# Autodesk Inventor assembly: RightMecanum-SubAssem01_MIR1
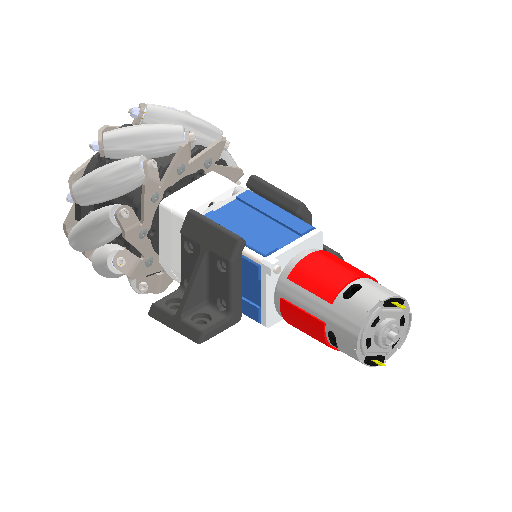
[picture p0: Inventor's stored thumbnail of the model, 512x512]
Saved by Autodesk Inventor 2024.1 (Build 281209000, 209)
## iProperties
Created: 2022-07-11
Part Number: RightMecanum-SubAssem01_MIR1
Document SubType Name: Assembly
Designer: dbt5238
Author: Dave
## Documents named in this file (9)
- E:\ChalkbotMechanical\Chalkbot1.0\Chassis\V1\RightMecanum-SubAssem01_MIR1.iam
- E:\ChalkbotMechanical\Chalkbot1.0\Chassis\V1\Motor and Gearbox STEP files\2 Stage HD - 57 Sport_MIR1.ipt
- E:\ChalkbotMechanical\Chalkbot1.0\Chassis\V1\Mechanum STEP files\am-3775a AndyMark RedLine Motor (1)_MIR1.ipt
- E:\ChalkbotMechanical\Chalkbot1.0\Chassis\V1\Motor and Gearbox STEP files\Hex Bore Mag Encoder Housing (217-6785)_MIR1.iam
- E:\ChalkbotMechanical\Chalkbot1.0\Chassis\V1\Motor and Gearbox STEP files\am-3791 - 3000 x 500 Hex Shaft_MIR1.ipt
- E:\ChalkbotMechanical\Chalkbot1.0\Chassis\V1\Motor Mounts_MIR1.ipt
- E:\ChalkbotMechanical\Chalkbot1.0\Chassis\V1\Shaft Spacers V2_MIR1.ipt
- E:\ChalkbotMechanical\Chalkbot1.0\Chassis\V1\Mechanum STEP files\am-3918L 4HD 500H Mecanum Right_MIR1.iam
- E:\ChalkbotMechanical\Chalkbot1.0\Chassis\V1\Motor and Gearbox STEP files\am-2986 FR8ZZ Hex Bearing_MIR1.ipt
## Components (15 placed, 8 different names)
1. 2 Stage HD - 57 Sport_MIR1:1 — Angle:1, Insert:4, Insert:7, Insert:6, Insert:9, Insert:8, Rigid:2, Cylindrical:1, Rotational:1
2. am-3775a AndyMark RedLine Motor (1)_MIR1:1 — Rigid:2
3. Hex Bore Mag Encoder Housing (217-6785)_MIR1:1 [sub-assembly] — Mate:4, Cylindrical:1, Rotational:1
4. am-3791 - 3000 x 500 Hex Shaft_MIR1:1 — Insert:4, Mate:6, Mate:5, Mate:9, Mate:8, Mate:12, Mate:11
5. Motor Mounts_MIR1:1 — Insert:7, Insert:6
6. Motor Mounts_MIR1:2 — Insert:9, Insert:8
7. Shaft Spacers V2_MIR1:1 — Rigid:3, Rigid:4
8. Shaft Spacers V2_MIR1:2 — Rigid:3, Rigid:5
9. Shaft Spacers V2_MIR1:3 — Rigid:4, Rigid:6
10. Shaft Spacers V2_MIR1:4 — Rigid:5, Rigid:7
11. Shaft Spacers V2_MIR1:5 — Mate:4, Rigid:6
12. Shaft Spacers V2_MIR1:6 — Rigid:7, Rigid:8
13. Shaft Spacers V2_MIR1:7 — Mate:6, Mate:5, Mate:7, Rigid:8
14. am-3918L 4HD 500H Mecanum Right_MIR1:1 [sub-assembly] — Mate:9, Mate:8, Mate:7, Mate:10
15. am-2986 FR8ZZ Hex Bearing_MIR1:1 — Mate:12, Mate:11, Mate:10
## Relationships (24: Mate 9, WeldJoint 7, Insert 5, Angle 1, CylindricalJoint 1, RevoluteJoint 1)
- Angle:1 (0 deg): 2 Stage HD - 57 Sport_MIR1:1
- Insert:4: 2 Stage HD - 57 Sport_MIR1:1 ↔ am-3791 - 3000 x 500 Hex Shaft_MIR1:1
- Insert:7: 2 Stage HD - 57 Sport_MIR1:1 ↔ Motor Mounts_MIR1:1
- Insert:6: 2 Stage HD - 57 Sport_MIR1:1 ↔ Motor Mounts_MIR1:1
- Insert:9: 2 Stage HD - 57 Sport_MIR1:1 ↔ Motor Mounts_MIR1:2
- Insert:8: 2 Stage HD - 57 Sport_MIR1:1 ↔ Motor Mounts_MIR1:2
- Mate:4: Hex Bore Mag Encoder Housing (217-6785)_MIR1:1 ↔ Shaft Spacers V2_MIR1:5
- Mate:6 (0.15 mm): am-3791 - 3000 x 500 Hex Shaft_MIR1:1 ↔ Shaft Spacers V2_MIR1:7
- Mate:5 (0.15 mm): am-3791 - 3000 x 500 Hex Shaft_MIR1:1 ↔ Shaft Spacers V2_MIR1:7
- Mate:9: am-3791 - 3000 x 500 Hex Shaft_MIR1:1 ↔ am-3918L 4HD 500H Mecanum Right_MIR1:1
- Mate:8: am-3791 - 3000 x 500 Hex Shaft_MIR1:1 ↔ am-3918L 4HD 500H Mecanum Right_MIR1:1
- Mate:7: Shaft Spacers V2_MIR1:7 ↔ am-3918L 4HD 500H Mecanum Right_MIR1:1
- Mate:12: am-3791 - 3000 x 500 Hex Shaft_MIR1:1 ↔ am-2986 FR8ZZ Hex Bearing_MIR1:1
- Mate:11: am-3791 - 3000 x 500 Hex Shaft_MIR1:1 ↔ am-2986 FR8ZZ Hex Bearing_MIR1:1
- Mate:10: am-3918L 4HD 500H Mecanum Right_MIR1:1 ↔ am-2986 FR8ZZ Hex Bearing_MIR1:1
- Rigid:2 [WeldJoint]: 2 Stage HD - 57 Sport_MIR1:1 ↔ am-3775a AndyMark RedLine Motor (1)_MIR1:1
- Cylindrical:1: 2 Stage HD - 57 Sport_MIR1:1 ↔ Hex Bore Mag Encoder Housing (217-6785)_MIR1:1
- Rotational:1 [RevoluteJoint]: 2 Stage HD - 57 Sport_MIR1:1 ↔ Hex Bore Mag Encoder Housing (217-6785)_MIR1:1
- Rigid:3 [WeldJoint]: Shaft Spacers V2_MIR1:1 ↔ Shaft Spacers V2_MIR1:2
- Rigid:4 [WeldJoint]: Shaft Spacers V2_MIR1:1 ↔ Shaft Spacers V2_MIR1:3
- Rigid:5 [WeldJoint]: Shaft Spacers V2_MIR1:2 ↔ Shaft Spacers V2_MIR1:4
- Rigid:6 [WeldJoint]: Shaft Spacers V2_MIR1:3 ↔ Shaft Spacers V2_MIR1:5
- Rigid:7 [WeldJoint]: Shaft Spacers V2_MIR1:4 ↔ Shaft Spacers V2_MIR1:6
- Rigid:8 [WeldJoint]: Shaft Spacers V2_MIR1:6 ↔ Shaft Spacers V2_MIR1:7
